# Autodesk Inventor assembly: Receiver Casing
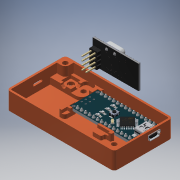
[picture p0: Inventor's stored thumbnail of the model, 180x180]
Saved by Autodesk Inventor 2019.4 (Build 234330000, 330)
## iProperties
Created: 2019-07-14
Part Number: Receiver Casing
Document SubType Name: Assembly
Designer: Petar
Author: Petar
## Documents named in this file (5)
- D:\OMG\E-Board\CAD\Inventor\Remote\Open Source nRF Remote\Receiver Casing.iam
- D:\OMG\E-Board\CAD\Inventor\Remote\Open Source nRF Remote\Receiver-casing.ipt
- D:\OMG\E-Board\CAD\Inventor\Remote\Open Source nRF Remote\Receiver-lid.ipt
- D:\OMG\E-Board\CAD\Inventor\Electrical Components\nRF24L01+_enhanced.ipt
- D:\OMG\E-Board\CAD\Inventor\Electrical Components\Arduino Nano\arduino nano.iam
## Components (4 placed, 4 different names)
1. Receiver-casing:1 — Rigid:1, Rigid:2
2. Receiver-lid:1 — Rigid:1
3. nRF24L01+_enhanced:1
4. arduino nano:1 [sub-assembly] — Rigid:2
## Relationships (2: WeldJoint 2)
- Rigid:1 [WeldJoint]: Receiver-casing:1 ↔ Receiver-lid:1
- Rigid:2 [WeldJoint]: Receiver-casing:1 ↔ arduino nano:1
